# Autodesk Inventor assembly: HubMotor
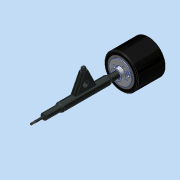
[picture p0: Inventor's stored thumbnail of the model, 180x180]
Saved by Autodesk Inventor 2015 (Build 190159000, 159)
## iProperties
Created: 2015-12-24
Part Number: HubMotor
Document SubType Name: Assembly
Designer: Raphael
Author: Raphael
## Documents named in this file (8)
- \\psf\Home\Documents\electric-skateboard\CAD\HubMotor\HubMotor.iam
- \\psf\Home\Documents\electric-skateboard\CAD\Paris Trucks.ipt
- \\psf\Home\Documents\electric-skateboard\CAD\HubMotor\GearboxAssembly.iam
- \\psf\Home\Documents\electric-skateboard\CAD\HubMotor\Mount.ipt
- \\psf\Home\Documents\electric-skateboard\CAD\HubMotor\M8Bearing.ipt
- \\psf\Home\Documents\electric-skateboard\CAD\HubMotor\RingGear.ipt
- \\psf\Home\Documents\electric-skateboard\CAD\HubMotor\BigBearing.ipt
- \\psf\Home\Documents\electric-skateboard\CAD\HubMotor\Wheel.ipt
## Components (8 placed, 7 different names)
1. Paris Trucks:1 — Mate:1, Mate:2, Flush:1, Mate:8
2. GearboxAssembly:1 [sub-assembly] — Mate:2, Mate:3, Mate:4, Mate:5, Mate:6, Mate:7, Mate:8, Flush:2
3. Mount:1 — Mate:1, Mate:6, Mate:7, Mate:9, Mate:10
4. M8Bearing:1 — Mate:3, Mate:4
5. M8Bearing:2 — Mate:5, Flush:1
6. RingGear:1 — Mate:11, Flush:2
7. BigBearing:1 — Mate:9, Mate:10, Mate:12, Flush:3
8. Wheel:1 — Mate:11, Mate:12, Flush:3
## Relationships (15: Mate 12, Flush 3)
- Mate:1: Paris Trucks:1 ↔ Mount:1
- Mate:2: Paris Trucks:1 ↔ GearboxAssembly:1
- Mate:3: GearboxAssembly:1 ↔ M8Bearing:1
- Mate:4: GearboxAssembly:1 ↔ M8Bearing:1
- Mate:5: GearboxAssembly:1 ↔ M8Bearing:2
- Mate:6: GearboxAssembly:1 ↔ Mount:1
- Mate:7: GearboxAssembly:1 ↔ Mount:1
- Flush:1: Paris Trucks:1 ↔ M8Bearing:2
- Mate:8 (1 mm): Paris Trucks:1 ↔ GearboxAssembly:1
- Mate:9: Mount:1 ↔ BigBearing:1
- Mate:10: Mount:1 ↔ BigBearing:1
- Mate:11: RingGear:1 ↔ Wheel:1
- Mate:12: BigBearing:1 ↔ Wheel:1
- Flush:2: GearboxAssembly:1 ↔ RingGear:1
- Flush:3: BigBearing:1 ↔ Wheel:1
